# Autodesk Inventor assembly: anhaenger_gesamt
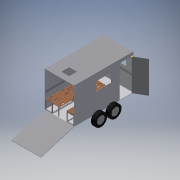
[picture p0: Inventor's stored thumbnail of the model, 180x180]
Saved by Autodesk Inventor 2018 (Build 220112000, 112)
## iProperties
Created: 2020-03-17
Part Number: anhaenger_gesamt
Material: Generisch
Document SubType Name: Assembly
Designer: wepet
Author: wepet
## Documents named in this file (16)
- C:\Users\wepet\Downloads\anhaenger\current\gesamt\anhaenger_gesamt.iam
- C:\Users\wepet\Downloads\anhaenger\current\details\reifen\reifen_achse.iam
- C:\Users\wepet\Downloads\anhaenger\current\details\chassis\Koffer_dach.ipt
- C:\Users\wepet\Downloads\anhaenger\current\details\chassis\Koffer_klappe.ipt
- C:\Users\wepet\Downloads\anhaenger\current\details\chassis\Koffer_leer.ipt
- C:\Users\wepet\Downloads\anhaenger\current\details\chassis\deichsel.ipt
- C:\Users\wepet\Downloads\anhaenger\current\details\chassis\Koffer_tuer.ipt
- C:\Users\wepet\Downloads\anhaenger\current\details\schienen\Koffer_ankerschiene_2m.ipt
- C:\Users\wepet\Downloads\anhaenger\current\details\schienen\Koffer_ankerschiene_3m.ipt
- C:\Users\wepet\Downloads\anhaenger\current\details\schienen\Koffer_ankerschiene_15m.ipt
- C:\Users\wepet\Downloads\anhaenger\current\details\schienen\Boden_airline_eckig.ipt
- C:\Users\wepet\Downloads\anhaenger\current\details\schienen\Boden_airline_rund.ipt
- C:\Users\wepet\Downloads\anhaenger\current\details\bett\bett_V1\bett_V1.iam
- C:\Users\wepet\Downloads\anhaenger\current\details\bett\bett_V2\bett_V2_doppelt.iam
- C:\Users\wepet\Downloads\anhaenger\current\details\bett\bett_V3\bett_V3_doppelt1.iam
- C:\Users\wepet\Downloads\anhaenger\current\details\bett\bett_V3\bett_V3_doppelt2.iam
## Components (19 placed, 18 different names)
1. reifen_achse:1 [sub-assembly] — Passend:4, Tangential:1, Passend:5, Tangential:3
2. reifen_achse:2 [sub-assembly] — Passend:3, Tangential:2, Passend:5
3. Koffer_dach:1 — Passend:2, Fluchtend:3, Fluchtend:4
4. Koffer_klappe:1 — Drehbar:1
5. Koffer_leer:1 — Fluchtend:1, Fluchtend:2, Passend:1, Passend:2, Fluchtend:3, Fluchtend:4, Drehbar:1, Passend:3, Passend:4, Tangential:1, Tangential:2, Tangential:3, Passend:6, Passend:7, Fluchtend:5, Drehbar:2, Passend:10, Fluchtend:7, Passend:11, Fluchtend:8, Passend:12, Passend:13, Passend:14, Passend:16, Passend:18, Passend:21, Passend:22, Passend:23, Passend:24, Passend:26, Passend:27, Fluchtend:11, Passend:29, Passend:31, Fluchtend:13, Fluchtend:15, Fluchtend:16, Fluchtend:17, Passend:32, Passend:33, Passend:34, Passend:35, Fluchtend:18, Fluchtend:19, Passend:36, Passend:37, Passend:38, Passend:39, Fluchtend:20, Fluchtend:21
6. deichsel:1 — Passend:6, Passend:7, Fluchtend:5
7. Koffer_tuer:1 — Drehbar:2
8. Koffer_ankerschiene_3m:L — Passend:11, Fluchtend:8, Passend:12, Fluchtend:9, Fluchtend:10
9. Koffer_ankerschiene_2m:R — Passend:10, Fluchtend:7, Fluchtend:9
10. Koffer_ankerschiene_15m:V — Passend:13, Fluchtend:10, Passend:14
11. Boden_airline_eckig:L — Passend:18, Passend:22, Fluchtend:16
12. Boden_airline_eckig:R — Passend:16, Passend:21, Fluchtend:17
13. Boden_airline_rund:1 — Passend:23, Passend:24, Fluchtend:15
14. bett_V1:L [sub-assembly] — Passend:26, Passend:27, Fluchtend:11
15. bett_V1:R [sub-assembly] — Passend:29, Passend:31, Fluchtend:13
16. bett_V2:L [sub-assembly] — Passend:33, Passend:34, Fluchtend:18
17. bett_V2:R [sub-assembly] — Passend:32, Passend:35, Fluchtend:19
18. bett_V3:L [sub-assembly] — Passend:36, Passend:38, Fluchtend:21
19. bett_V3:R [sub-assembly] — Passend:37, Passend:39, Fluchtend:20
## Relationships (53: Mate 30, Flush 18, Tangent 3, RevoluteJoint 2)
- Fluchtend:1 [Flush]: Koffer_leer:1
- Fluchtend:2 [Flush] (75 mm): Koffer_leer:1
- Passend:1 [Mate]: Koffer_leer:1
- Passend:2 [Mate]: Koffer_dach:1 ↔ Koffer_leer:1
- Fluchtend:3 [Flush]: Koffer_dach:1 ↔ Koffer_leer:1
- Fluchtend:4 [Flush]: Koffer_dach:1 ↔ Koffer_leer:1
- Drehbar:1 [RevoluteJoint]: Koffer_klappe:1 ↔ Koffer_leer:1
- Passend:3 [Mate] (3.5 mm): reifen_achse:2 ↔ Koffer_leer:1
- Passend:4 [Mate] (3.5 mm): reifen_achse:1 ↔ Koffer_leer:1
- Tangential:1 (-21.5 mm): reifen_achse:1 ↔ Koffer_leer:1
- Tangential:2 (-21.5 mm): reifen_achse:2 ↔ Koffer_leer:1
- Passend:5 [Mate] (75 mm): reifen_achse:1 ↔ reifen_achse:2
- Tangential:3 (-119 mm): reifen_achse:1 ↔ Koffer_leer:1
- Passend:6 [Mate]: Koffer_leer:1 ↔ deichsel:1
- Passend:7 [Mate]: Koffer_leer:1 ↔ deichsel:1
- Fluchtend:5 [Flush] (-67.5 mm): Koffer_leer:1 ↔ deichsel:1
- Drehbar:2 [RevoluteJoint]: Koffer_leer:1 ↔ Koffer_tuer:1
- Passend:10 [Mate]: Koffer_leer:1 ↔ Koffer_ankerschiene_2m:R
- Fluchtend:7 [Flush] (2 mm): Koffer_leer:1 ↔ Koffer_ankerschiene_2m:R
- Passend:11 [Mate]: Koffer_leer:1 ↔ Koffer_ankerschiene_3m:L
- Fluchtend:8 [Flush] (-2 mm): Koffer_leer:1 ↔ Koffer_ankerschiene_3m:L
- Passend:12 [Mate] (73.5 mm): Koffer_leer:1 ↔ Koffer_ankerschiene_3m:L
- Fluchtend:9 [Flush]: Koffer_ankerschiene_3m:L ↔ Koffer_ankerschiene_2m:R
- Passend:13 [Mate]: Koffer_leer:1 ↔ Koffer_ankerschiene_15m:V
- Fluchtend:10 [Flush]: Koffer_ankerschiene_3m:L ↔ Koffer_ankerschiene_15m:V
- Passend:14 [Mate]: Koffer_leer:1 ↔ Koffer_ankerschiene_15m:V
- Passend:16 [Mate]: Koffer_leer:1 ↔ Boden_airline_eckig:R
- Passend:18 [Mate]: Koffer_leer:1 ↔ Boden_airline_eckig:L
- Passend:21 [Mate] (38 mm): Koffer_leer:1 ↔ Boden_airline_eckig:R
- Passend:22 [Mate] (38 mm): Koffer_leer:1 ↔ Boden_airline_eckig:L
- Passend:23 [Mate]: Koffer_leer:1 ↔ Boden_airline_rund:1
- Passend:24 [Mate] (72.5 mm): Koffer_leer:1 ↔ Boden_airline_rund:1
- Passend:26 [Mate]: Koffer_leer:1 ↔ bett_V1:L
- Passend:27 [Mate]: Koffer_leer:1 ↔ bett_V1:L
- Fluchtend:11 [Flush]: Koffer_leer:1 ↔ bett_V1:L
- Passend:29 [Mate]: Koffer_leer:1 ↔ bett_V1:R
- Passend:31 [Mate]: Koffer_leer:1 ↔ bett_V1:R
- Fluchtend:13 [Flush]: Koffer_leer:1 ↔ bett_V1:R
- Fluchtend:15 [Flush] (10 mm): Koffer_leer:1 ↔ Boden_airline_rund:1
- Fluchtend:16 [Flush] (10 mm): Koffer_leer:1 ↔ Boden_airline_eckig:L
- Fluchtend:17 [Flush] (10 mm): Koffer_leer:1 ↔ Boden_airline_eckig:R
- Passend:32 [Mate]: Koffer_leer:1 ↔ bett_V2:R
- Passend:33 [Mate]: Koffer_leer:1 ↔ bett_V2:L
- Passend:34 [Mate]: Koffer_leer:1 ↔ bett_V2:L
- Passend:35 [Mate]: Koffer_leer:1 ↔ bett_V2:R
- Fluchtend:18 [Flush]: Koffer_leer:1 ↔ bett_V2:L
- Fluchtend:19 [Flush]: Koffer_leer:1 ↔ bett_V2:R
- Passend:36 [Mate]: Koffer_leer:1 ↔ bett_V3:L
- Passend:37 [Mate]: Koffer_leer:1 ↔ bett_V3:R
- Passend:38 [Mate]: Koffer_leer:1 ↔ bett_V3:L
- Passend:39 [Mate]: Koffer_leer:1 ↔ bett_V3:R
- Fluchtend:20 [Flush]: Koffer_leer:1 ↔ bett_V3:R
- Fluchtend:21 [Flush]: Koffer_leer:1 ↔ bett_V3:L
